# Autodesk Inventor assembly: bellows_latest
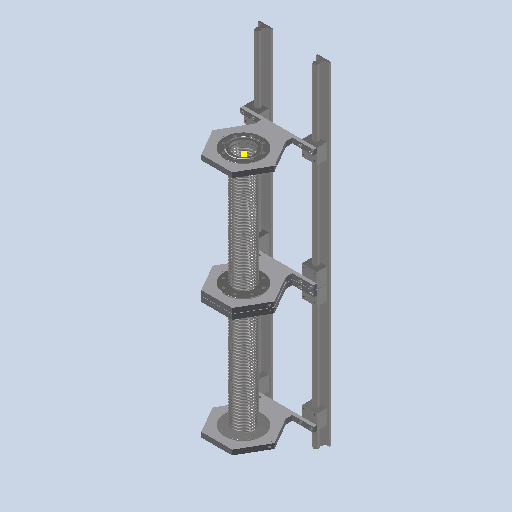
[picture p0: Inventor's stored thumbnail of the model, 512x512]
Saved by Autodesk Inventor 2026.3 (Build 303398000, 398)
## iProperties
Created: 2026-06-04
Part Number: bellows_latest
Document SubType Name: Assembly
Designer: shusu
Author: shusu
## Documents named in this file (3)
- C:\Users\shusu\aklab_pihti\PIHTI\bellows\bellows.iam
- C:\Users\shusu\aklab_pihti\PIHTI\bellows\rail.ipt
- C:\Users\shusu\aklab_pihti\PIHTI\bellows\bellows_2.iam
## Components (4 placed, 2 different names)
1. rail:1 — 挿入:2
2. rail:2 — 挿入:1
3. bellows_2:1 [sub-assembly] — 挿入:1, 挿入:2, メイト:1
4. bellows_2:2 [sub-assembly] — メイト:1
## Relationships (3: Insert 2, Mate 1)
- 挿入:1 [Insert] (-800 mm): rail:2 ↔ bellows_2:1
- 挿入:2 [Insert] (-800 mm): rail:1 ↔ bellows_2:1
- メイト:1 [Mate]: bellows_2:1 ↔ bellows_2:2
